# Autodesk Inventor assembly: Worm-Drive-Gearbox-16to1
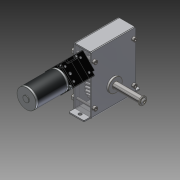
[picture p0: Inventor's stored thumbnail of the model, 180x180]
Saved by Autodesk Inventor 2014 SP1 (Build 180222100, 222)
## iProperties
Created: 2014-01-05
Part Number: Worm-Drive-Gearbox-16to1
Document SubType Name: Assembly
Designer: Arpan
Mass: 1215.63 g
Surface Area: 1943.18 cm^2
Volume: 378.034 cm^3
Density: 3.21566 g/cm^3
Author: Mark
Title: Worm Drive Gearbox 16to1.STEP
Description: STEP AP214
Creation Date: 2012-01-19
Sending System: SolidWorks 2010
Preprocessor: SwSTEP 2.0
Author: Arpan
## Documents named in this file (23)
- C:\Users\Moses\Documents\GitHub\2014buildCAD\Shooter\Worm-Drive-Gearbox-16to1.iam
- C:\Users\Moses\Documents\GitHub\2014buildCAD\Imported Components\Worm-Drive-Gearbox-16to1\FR6ZZ Bearing.ipt
- C:\Users\Moses\Documents\GitHub\2014buildCAD\Imported Components\Worm-Drive-Gearbox-16to1\Socket Head Cap Screw_AI_HX-SHCS 0.19-32x0.375x0.375-C.ipt
- C:\Users\Moses\Documents\GitHub\2014buildCAD\Imported Components\Worm-Drive-Gearbox-16to1\washer 0.25_Preferred Narrow FW 0.25.ipt
- C:\Users\Moses\Documents\GitHub\2014buildCAD\Imported Components\Worm-Drive-Gearbox-16to1\Motor mount.ipt
- C:\Users\Moses\Documents\GitHub\2014buildCAD\Imported Components\Worm-Drive-Gearbox-16to1\BHCS 0.25-20x0.625_SBHCSCREW 0.25-20x0.625-HX-C.ipt
- C:\Users\Moses\Documents\GitHub\2014buildCAD\Imported Components\Worm-Drive-Gearbox-16to1\500 hex to 8mm adapter.ipt
- C:\Users\Moses\Documents\GitHub\2014buildCAD\Imported Components\Worm-Drive-Gearbox-16to1\10-32 Nylock Nut 1_90631A411.ipt
- C:\Users\Moses\Documents\GitHub\2014buildCAD\Imported Components\Worm-Drive-Gearbox-16to1\LH Helical gear 12DP 32T 10HA 14.5PA 0.5FW_Inch - LH Helical gear 12DP 32T 10HA 14.5PA 0.5FW ---32N3.0H2.0L0.5N.ipt
- C:\Users\Moses\Documents\GitHub\2014buildCAD\Imported Components\Worm-Drive-Gearbox-16to1\SHCS 10-32x1.75_HX-SHCS 0.19-32x1.75x0.875-C.ipt
- C:\Users\Moses\Documents\GitHub\2014buildCAD\Imported Components\Worm-Drive-Gearbox-16to1\worm shaft.ipt
- C:\Users\Moses\Documents\GitHub\2014buildCAD\Imported Components\Worm-Drive-Gearbox-16to1\worm.ipt
- C:\Users\Moses\Documents\GitHub\2014buildCAD\Imported Components\Worm-Drive-Gearbox-16to1\worm spacer.ipt
- C:\Users\Moses\Documents\GitHub\2014buildCAD\Imported Components\Worm-Drive-Gearbox-16to1\End plate.ipt
- C:\Users\Moses\Documents\GitHub\2014buildCAD\Imported Components\Worm-Drive-Gearbox-16to1\o Plate.ipt
- C:\Users\Moses\Documents\GitHub\2014buildCAD\Imported Components\Worm-Drive-Gearbox-16to1\8mm spacer.ipt
- C:\Users\Moses\Documents\GitHub\2014buildCAD\Imported Components\Worm-Drive-Gearbox-16to1\worm gear ring.ipt
- C:\Users\Moses\Documents\GitHub\2014buildCAD\Imported Components\Worm-Drive-Gearbox-16to1\FR8ZZ Bearing.ipt
- C:\Users\Moses\Documents\GitHub\2014buildCAD\Imported Components\Worm-Drive-Gearbox-16to1\encoder bracket.ipt
- C:\Users\Moses\Documents\GitHub\2014buildCAD\Imported Components\Worm-Drive-Gearbox-16to1\PIN  0.1875x.75_SPS 0.1875x0.75.ipt
- C:\Users\Moses\Documents\GitHub\2014buildCAD\Imported Components\Worm-Drive-Gearbox-16to1\output shaft.ipt
- C:\Users\Moses\Documents\GitHub\2014buildCAD\Imported Components\Worm-Drive-Gearbox-16to1\Plate.ipt
- C:\Users\Moses\Documents\GitHub\2014buildCAD\Shooter\217-2 Stage Versaplanetary STEP.iam
## Components (33 placed, 33 different names)
1. FR6ZZ Bearing_1 — Insert:1, Insert:11, Insert:13
2. Socket Head Cap Screw_AI_HX-SHCS 0.19-32x0.375x0.375-C_2 — Insert:6
3. washer 0.25_Preferred Narrow FW 0.25_3 — Insert:2, Insert:3
4. Socket Head Cap Screw_AI_HX-SHCS 0.19-32x0.375x0.375-C_5 — Insert:5
5. Motor mount_6 — Mate:1, Mate:2, Mate:3, Mate:7, Flush:5, Mate:20
6. BHCS 0.25-20x0.625_SBHCSCREW 0.25-20x0.625-HX-C_7 — Insert:2, Rotation:2
7. 500 hex to 8mm adapter_8
8. 10-32 Nylock Nut 1_90631A411_9 — Insert:8
9. LH Helical gear 12DP 32T 10HA 14.5PA 0.5FW_Inch - LH Helical gear 12DP 32T 10HA 14.5PA 0.5FW ---32N3.0H2.0L0.5N_10 — Mate:14, Mate:15, Mate:16, Rotation:1, Tangent:1
10. SHCS 10-32x1.75_HX-SHCS 0.19-32x1.75x0.875-C_11
11. worm shaft_12 — Insert:11, Mate:12, Mate:13, Rotation:1, Rotation:3
12. 10-32 Nylock Nut 1_90631A411_13 — Insert:9
13. worm_14 — Mate:9, Mate:11, Insert:12, Mate:13
14. SHCS 10-32x1.75_HX-SHCS 0.19-32x1.75x0.875-C_15
15. worm spacer_16 — Mate:11, Insert:12, Insert:13, Mate:12
16. 10-32 Nylock Nut 1_90631A411_17 — Insert:10
17. End plate_18 — Insert:1, Flush:3, Flush:4, Mate:19
18. SHCS 10-32x1.75_HX-SHCS 0.19-32x1.75x0.875-C_19
19. worm spacer_20 — Mate:8, Mate:9, Rotation:3
20. 10-32 Nylock Nut 1_90631A411_21 — Insert:7
21. o Plate_22 — Insert:4, Insert:7, Insert:8, Insert:9, Insert:10, Mate:4, Mate:5, Mate:6, Flush:1, Flush:2, Flush:4, Mate:19, Mate:20
22. SHCS 10-32x1.75_HX-SHCS 0.19-32x1.75x0.875-C_23
23. 8mm spacer_24 — Mate:7, Mate:8
24. worm gear ring_25 — Insert:15
25. FR8ZZ Bearing_26 — Insert:14, Insert:15, Mate:14, Mate:15
26. encoder bracket_27 — Insert:5, Insert:6, Mate:4, Mate:5, Mate:6
27. PIN  0.1875x.75_SPS 0.1875x0.75_28 — Mate:16, Mate:18, Tangent:1
28. worm gear ring_29 — Insert:16
29. FR8ZZ Bearing_30 — Insert:4, Insert:16, Mate:17
30. output shaft_31 — Insert:3, Flush:1, Mate:17, Mate:18, Rotation:2
31. Plate_32 — Insert:14, Flush:2, Flush:3, Flush:5
32. PIN  0.1875x.75_SPS 0.1875x0.75_33
33. 217-2 Stage Versaplanetary STEP:1 [sub-assembly] — Mate:1, Mate:2, Mate:3
## Relationships (44: Mate 19, Insert 16, Flush 5, RelateRotation 3, Tangent 1)
- Mate:1: Motor mount_6 ↔ 217-2 Stage Versaplanetary STEP:1
- Mate:2: Motor mount_6 ↔ 217-2 Stage Versaplanetary STEP:1
- Mate:3: Motor mount_6 ↔ 217-2 Stage Versaplanetary STEP:1
- Insert:1: FR6ZZ Bearing_1 ↔ End plate_18
- Insert:2: washer 0.25_Preferred Narrow FW 0.25_3 ↔ BHCS 0.25-20x0.625_SBHCSCREW 0.25-20x0.625-HX-C_7
- Insert:3: washer 0.25_Preferred Narrow FW 0.25_3 ↔ output shaft_31
- Insert:4: o Plate_22 ↔ FR8ZZ Bearing_30
- Insert:5: Socket Head Cap Screw_AI_HX-SHCS 0.19-32x0.375x0.375-C_5 ↔ encoder bracket_27
- Insert:6: Socket Head Cap Screw_AI_HX-SHCS 0.19-32x0.375x0.375-C_2 ↔ encoder bracket_27
- Insert:7: 10-32 Nylock Nut 1_90631A411_21 ↔ o Plate_22
- Insert:8: 10-32 Nylock Nut 1_90631A411_9 ↔ o Plate_22
- Insert:9: 10-32 Nylock Nut 1_90631A411_13 ↔ o Plate_22
- Insert:10: 10-32 Nylock Nut 1_90631A411_17 ↔ o Plate_22
- Mate:4: o Plate_22 ↔ encoder bracket_27
- Mate:5: o Plate_22 ↔ encoder bracket_27
- Mate:6: o Plate_22 ↔ encoder bracket_27
- Mate:7: Motor mount_6 ↔ 8mm spacer_24
- Mate:8: worm spacer_20 ↔ 8mm spacer_24
- Mate:9: worm_14 ↔ worm spacer_20
- Mate:11: worm_14 ↔ worm spacer_16
- Insert:11 (-0.7747 mm): FR6ZZ Bearing_1 ↔ worm shaft_12
- Insert:12: worm_14 ↔ worm spacer_16
- Insert:13: FR6ZZ Bearing_1 ↔ worm spacer_16
- Mate:12: worm shaft_12 ↔ worm spacer_16
- Mate:13: worm shaft_12 ↔ worm_14
- Insert:14: FR8ZZ Bearing_26 ↔ Plate_32
- Insert:15 (0.0127 mm): worm gear ring_25 ↔ FR8ZZ Bearing_26
- Insert:16 (0.0127 mm): worm gear ring_29 ↔ FR8ZZ Bearing_30
- Mate:14 (12.7127 mm): LH Helical gear 12DP 32T 10HA 14.5PA 0.5FW_Inch - LH Helical gear 12DP 32T 10HA 14.5PA 0.5FW ---32N3.0H2.0L0.5N_10 ↔ FR8ZZ Bearing_26
- Mate:15: LH Helical gear 12DP 32T 10HA 14.5PA 0.5FW_Inch - LH Helical gear 12DP 32T 10HA 14.5PA 0.5FW ---32N3.0H2.0L0.5N_10 ↔ FR8ZZ Bearing_26
- Mate:16: LH Helical gear 12DP 32T 10HA 14.5PA 0.5FW_Inch - LH Helical gear 12DP 32T 10HA 14.5PA 0.5FW ---32N3.0H2.0L0.5N_10 ↔ PIN  0.1875x.75_SPS 0.1875x0.75_28
- Rotation:1 [RelateRotation] (0.0625 ul): LH Helical gear 12DP 32T 10HA 14.5PA 0.5FW_Inch - LH Helical gear 12DP 32T 10HA 14.5PA 0.5FW ---32N3.0H2.0L0.5N_10 ↔ worm shaft_12
- Flush:1 (-20.0025 mm): o Plate_22 ↔ output shaft_31
- Mate:17: FR8ZZ Bearing_30 ↔ output shaft_31
- Mate:18: PIN  0.1875x.75_SPS 0.1875x0.75_28 ↔ output shaft_31
- Tangent:1 (-1.27 mm): LH Helical gear 12DP 32T 10HA 14.5PA 0.5FW_Inch - LH Helical gear 12DP 32T 10HA 14.5PA 0.5FW ---32N3.0H2.0L0.5N_10 ↔ PIN  0.1875x.75_SPS 0.1875x0.75_28
- Flush:2: o Plate_22 ↔ Plate_32
- Flush:3: End plate_18 ↔ Plate_32
- Flush:4: End plate_18 ↔ o Plate_22
- Mate:19: End plate_18 ↔ o Plate_22
- Flush:5: Motor mount_6 ↔ Plate_32
- Mate:20: Motor mount_6 ↔ o Plate_22
- Rotation:2 [RelateRotation] (1 ul): BHCS 0.25-20x0.625_SBHCSCREW 0.25-20x0.625-HX-C_7 ↔ output shaft_31
- Rotation:3 [RelateRotation] (1 ul): worm shaft_12 ↔ worm spacer_20
